# Autodesk Inventor assembly: modul top
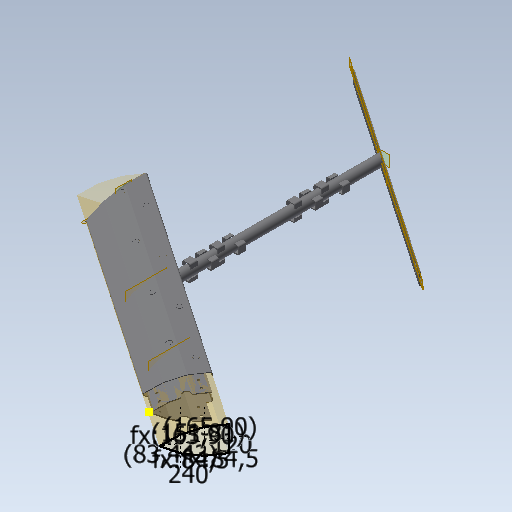
[picture p0: Inventor's stored thumbnail of the model, 512x512]
Saved by Autodesk Inventor 2020.1 (Build 241239000, 239)
## iProperties
Created: 2019-09-23
Part Number: modul top
Document SubType Name: Assembly
Designer: loppen
Mass: 34608.5 g
Surface Area: 22056.7 cm^2
Volume: 4408.73 cm^3
Density: 7.85 g/cm^3
Author: loppen
## Documents named in this file (20)
- Y:\trappe\modul top.iam
- Y:\trappe\model.ipt
- Y:\trappe\vange top.ipt
- Y:\trappe\top vange-endeplade.ipt
- Y:\trappe\baluster\stilladssøjle.iam
- Y:\trappe\baluster-fod.ipt
- Y:\trappe\håndfang\håndfang.iam
- Y:\trappe\trappestift skrå.ipt
- Y:\trappe\trappestift.ipt
- Y:\trappe\laske.ipt
- Y:\trappe\laske spejlet.ipt
- Y:\trappe\skot.ipt
- Y:\trappe\skot opad.ipt
- Y:\trappe\modul\AIP\FEA\d09v3y4ww.fins
- Y:\trappe\modul\AIP\FEA\d09v3y4ww.fsat
- Y:\trappe\modul\AIP\FEA\d09v3y4ww.ftes
- Y:\trappe\modul\AIP\FEA\d09v3y4ww.fwiz
- Y:\trappe\modul\AIP\FEA\d09v3y50g.fmsh
- Y:\trappe\modul\AIP\FEA\d09v3y50h.fres
- Y:\trappe\trappe.xlsx
## Components (18 placed, 12 different names)
1. model:1 — Flush:1, Flush:2, Flush:3, Flush:4, Flush:5, Flush:6, Flush:7, Flush:8
2. vange top:1 — Flush:1, Flush:2, Flush:3, Flush:4, Flush:5, Flush:6, Flush:7, Flush:8, Mate:1, Mate:2, Flush:9, Flush:10, Mate:4, Flush:11, Mate:8, Mate:9, Mate:10, Mate:11, Mate:12, Mate:13, Mate:14, Mate:15, Angle:2, Angle:3, Angle:4, Angle:5, Angle:6, Angle:7, Angle:8, Flush:12, Flush:13, Flush:14, Flush:15, Mate:16, Mate:17, Mate:18, Mate:19, Mate:20, Mate:21, Mate:22, Mate:23, Mate:24, Mate:25, Mate:26, Mate:27, Mate:28, Mate:29, Flush:17
3. top vange-endeplade:1 — Mate:1
4. stilladssøjle:1 [sub-assembly] — Mate:2, Flush:9, Mate:3, Mate:5, Mate:6, Mate:7
5. baluster-fod:1 — Flush:10, Mate:3, Mate:4, Mate:5, Flush:16
6. håndfang:1 [sub-assembly] — Mate:6, Flush:11, Mate:7
7. trappestift skrå:1 — Mate:8, Angle:1, Mate:16
8. trappestift:1 — Mate:9, Angle:1, Angle:2, Flush:12
9. trappestift skrå:3 — Mate:10, Angle:3, Mate:17
10. trappestift:2 — Mate:11, Angle:4, Flush:13
11. trappestift skrå:5 — Mate:12, Angle:5, Mate:18
12. trappestift:3 — Mate:13, Angle:6, Flush:14
13. trappestift skrå:7 — Mate:14, Angle:7, Mate:19
14. trappestift:4 — Mate:15, Angle:8, Flush:15
15. laske:1 — Mate:20, Mate:21, Mate:22
16. laske spejlet:1 — Mate:23, Mate:24, Mate:25
17. skot:1 — Mate:26, Mate:27, Flush:16
18. skot opad:1 — Mate:28, Mate:29, Flush:17
## Relationships (54: Mate 29, Flush 17, Angle 8)
- Flush:1: model:1 ↔ vange top:1
- Flush:2: model:1 ↔ vange top:1
- Flush:3: model:1 ↔ vange top:1
- Flush:4: model:1 ↔ vange top:1
- Flush:5: model:1 ↔ vange top:1
- Flush:6: model:1 ↔ vange top:1
- Flush:7: model:1 ↔ vange top:1
- Flush:8: model:1 ↔ vange top:1
- Mate:1: vange top:1 ↔ top vange-endeplade:1
- Mate:2: vange top:1 ↔ stilladssøjle:1
- Flush:9: vange top:1 ↔ stilladssøjle:1
- Flush:10: vange top:1 ↔ baluster-fod:1
- Mate:3: stilladssøjle:1 ↔ baluster-fod:1
- Mate:4 (43.655 mm): vange top:1 ↔ baluster-fod:1
- Mate:5: stilladssøjle:1 ↔ baluster-fod:1
- Mate:6: stilladssøjle:1 ↔ håndfang:1
- Flush:11: vange top:1 ↔ håndfang:1
- Mate:7 (-90 mm): stilladssøjle:1 ↔ håndfang:1
- Mate:8: vange top:1 ↔ trappestift skrå:1
- Mate:9: vange top:1 ↔ trappestift:1
- Mate:10: vange top:1 ↔ trappestift skrå:3
- Mate:11: vange top:1 ↔ trappestift:2
- Mate:12: vange top:1 ↔ trappestift skrå:5
- Mate:13: vange top:1 ↔ trappestift:3
- Mate:14: vange top:1 ↔ trappestift skrå:7
- Mate:15: vange top:1 ↔ trappestift:4
- Angle:1 (0 deg): trappestift skrå:1 ↔ trappestift:1
- Angle:2 (0 deg): vange top:1 ↔ trappestift:1
- Angle:3 (0 deg): vange top:1 ↔ trappestift skrå:3
- Angle:4 (0 deg): vange top:1 ↔ trappestift:2
- Angle:5 (0 deg): vange top:1 ↔ trappestift skrå:5
- Angle:6 (0 deg): vange top:1 ↔ trappestift:3
- Angle:7 (0 deg): vange top:1 ↔ trappestift skrå:7
- Angle:8 (0 deg): vange top:1 ↔ trappestift:4
- Flush:12: vange top:1 ↔ trappestift:1
- Flush:13: vange top:1 ↔ trappestift:2
- Flush:14: vange top:1 ↔ trappestift:3
- Flush:15: vange top:1 ↔ trappestift:4
- Mate:16: vange top:1 ↔ trappestift skrå:1
- Mate:17: vange top:1 ↔ trappestift skrå:3
- Mate:18: vange top:1 ↔ trappestift skrå:5
- Mate:19: vange top:1 ↔ trappestift skrå:7
- Mate:20: vange top:1 ↔ laske:1
- Mate:21: vange top:1 ↔ laske:1
- Mate:22 (32.5 mm): vange top:1 ↔ laske:1
- Mate:23: vange top:1 ↔ laske spejlet:1
- Mate:24: vange top:1 ↔ laske spejlet:1
- Mate:25 (32.5 mm): vange top:1 ↔ laske spejlet:1
- Mate:26: vange top:1 ↔ skot:1
- Mate:27 (1.659 mm): vange top:1 ↔ skot:1
- Flush:16 (-345.087 mm): baluster-fod:1 ↔ skot:1
- Mate:28: vange top:1 ↔ skot opad:1
- Mate:29: vange top:1 ↔ skot opad:1
- Flush:17 (13.5 mm): vange top:1 ↔ skot opad:1
## Named parameters: sa_0 = 0, sa_1 = 0, sa_2 = -250000, trappestifter_dia = 25 mm, trappestifter_laengde = 228 mm, perforeringsbredde = 6 mm, perforeringshulprocent = 80 mm, perforeringshullaengde = 62.8 mm, perforeringsoffset = 8 mm, perforeringsoffset_top = 8 mm, perforeringsoffset_bund = 8 mm, laskehul_dia = 13 mm, perforeringshullaengde_bund = 61.6 mm, perforeringshullaengde_top = 61 mm, trappestifter_huldia = 25.8 mm, trappestifter_skraa_huldia = 26.6 mm, håndfang_offset_fra_top = 70 mm, haandfang_offset_fra_top = 90 mm, trappevinkel = 34.3 deg, balusterhul_udvidelse = 1 mm, pladetykkelse = 3 mm, trinbredde = 1884 mm, trinhoejde = 100 mm
note: some values were not read from the file. Shown as the stored number, unit unknown: "sa_0", "sa_1", "sa_2".
